# Autodesk Inventor assembly: Mixer
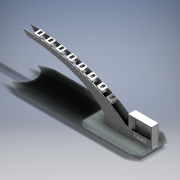
[picture p0: Inventor's stored thumbnail of the model, 180x180]
Saved by Autodesk Inventor 2016 (Build 200138000, 138)
## iProperties
Created: 2015-04-28
Part Number: Mixer
Document SubType Name: Assembly
Designer: Atok
Author: Atok
## Documents named in this file (7)
- C:\Users\Markus\Desktop\MakerBot Blade\Mixer.iam
- C:\Users\Markus\Desktop\MakerBot Blade\Block.ipt
- C:\Users\Markus\Desktop\MakerBot Blade\Blade.ipt
- C:\Users\Markus\Desktop\MakerBot Blade\Table.ipt
- C:\Users\Markus\Desktop\MakerBot Blade\DisplayBox.ipt
- C:\Users\Markus\Desktop\MakerBot Blade\Module.ipt
- C:\Users\Markus\Documents\Inventor\Content Center Files\R2016\en-US\M\M 6x12.ipt
## Components (20 placed, 6 different names)
1. Block:1 — Rigid:8, Rigid:5, Flush:4, Flush:5, Flush:6
2. Block:3 — Flush:1, Flush:2, Flush:3
3. Blade:1 — Rigid:8, Rigid:1, Rigid:16
4. Blade:2 — Rigid:5, Rigid:4, Rigid:6, Rigid:9, Rigid:10, Rigid:11, Rigid:12, Rigid:15, Rigid:13, Rigid:14, Rotational:3, Rotational:4, Rigid:17
5. Block:2 — Rigid:4
6. Block:4 — Rigid:16
7. Table:3 — Rigid:3
8. Table:2 — Rigid:2, Rigid:3
9. Table:1 — Rigid:1, Rigid:2
10. DisplayBox:1 — Rigid:6
11. Module:1 — Rigid:9
12. Module:2 — Rigid:10
13. Module:3 — Rigid:11
14. Module:4 — Rigid:12
15. Module:5 — Rigid:15
16. Module:6 — Rigid:13
17. Module:7 — Rigid:14
18. Module:8 — Rigid:17
19. M 6x12:2 — Rotational:3
20. M 6x12:1 — Rotational:4
## Relationships (24: WeldJoint 16, Flush 6, RevoluteJoint 2)
- Rigid:8 [WeldJoint]: Block:1 ↔ Blade:1
- Rigid:5 [WeldJoint]: Block:1 ↔ Blade:2
- Rigid:4 [WeldJoint]: Blade:2 ↔ Block:2
- Rigid:1 [WeldJoint]: Blade:1 ↔ Table:1
- Rigid:2 [WeldJoint]: Table:2 ↔ Table:1
- Rigid:3 [WeldJoint]: Table:3 ↔ Table:2
- Rigid:6 [WeldJoint]: Blade:2 ↔ DisplayBox:1
- Rigid:9 [WeldJoint]: Blade:2 ↔ Module:1
- Rigid:10 [WeldJoint]: Blade:2 ↔ Module:2
- Rigid:11 [WeldJoint]: Blade:2 ↔ Module:3
- Rigid:12 [WeldJoint]: Blade:2 ↔ Module:4
- Rigid:15 [WeldJoint]: Blade:2 ↔ Module:5
- Rigid:13 [WeldJoint]: Blade:2 ↔ Module:6
- Rigid:14 [WeldJoint]: Blade:2 ↔ Module:7
- Rotational:3 [RevoluteJoint]: Blade:2 ↔ M 6x12:2
- Rotational:4 [RevoluteJoint]: Blade:2 ↔ M 6x12:1
- Flush:1: Block:3
- Flush:2: Block:3
- Flush:3: Block:3
- Flush:4: Block:1
- Flush:5: Block:1
- Flush:6: Block:1
- Rigid:16 [WeldJoint]: Blade:1 ↔ Block:4
- Rigid:17 [WeldJoint]: Blade:2 ↔ Module:8
